# Autodesk Inventor assembly: DFPlayer Mini
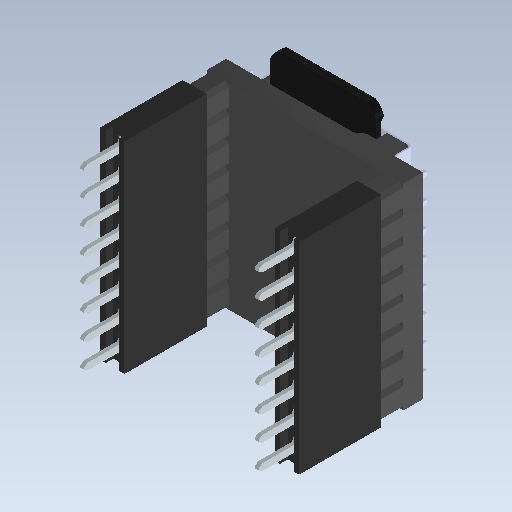
[picture p0: Inventor's stored thumbnail of the model, 512x512]
Saved by Autodesk Inventor 2021 (Build 250183000, 183)
## iProperties
Created: 2023-08-06
Part Number: DFPlayer Mini
Document SubType Name: Assembly
Designer: michal
Author: michal
## Documents named in this file (4)
- C:\Users\micha\OneDrive\Dokumenty\GitHub\escape_room_hw_v2\Enclosure\Commercial\DFPlayer Mini.iam
- C:\Users\micha\OneDrive\Dokumenty\GitHub\escape_room_hw_v2\Enclosure\Commercial\DFR0299.ipt
- C:\Users\micha\OneDrive\Dokumenty\GitHub\escape_room_hw_v2\Enclosure\Commercial\Micro SD Card.ipt
- C:\Users\micha\OneDrive\Dokumenty\GitHub\escape_room_hw_v2\Enclosure\Commercial\139343848-9-71071773\71071773.iam
## Components (4 placed, 3 different names)
1. DFR0299:1 — Mate:1, Mate:2, Flush:1, Flush:2, Mate:3, Flush:3, Flush:6
2. Micro SD Card:1 — Mate:1, Mate:2, Flush:1
3. 71071773:1 [sub-assembly] — Flush:2, Mate:3, Flush:3, Flush:4, Flush:5
4. 71071773:2 [sub-assembly] — Flush:4, Flush:5, Flush:6
## Relationships (9: Flush 6, Mate 3)
- Mate:1: DFR0299:1 ↔ Micro SD Card:1
- Mate:2: DFR0299:1 ↔ Micro SD Card:1
- Flush:1 (-2.5 mm): DFR0299:1 ↔ Micro SD Card:1
- Flush:2 (-0.107 mm): DFR0299:1 ↔ 71071773:1
- Mate:3: DFR0299:1 ↔ 71071773:1
- Flush:3 (-0.25 mm): DFR0299:1 ↔ 71071773:1
- Flush:4: 71071773:1 ↔ 71071773:2
- Flush:5: 71071773:1 ↔ 71071773:2
- Flush:6 (-0.107 mm): DFR0299:1 ↔ 71071773:2
